# Autodesk Inventor assembly: WCP-0897
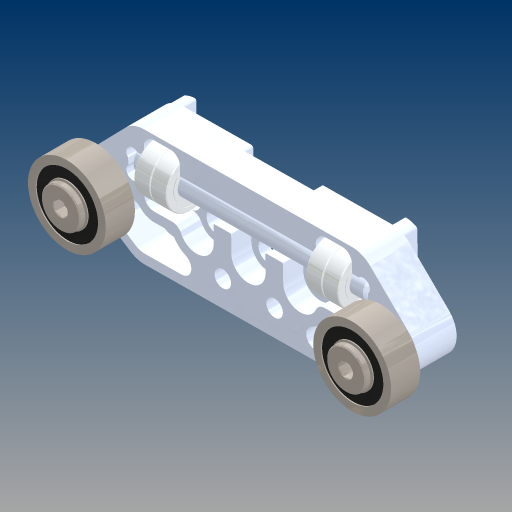
[picture p0: Inventor's stored thumbnail of the model, 512x512]
Saved by Autodesk Inventor 2024.3 (Build 283343000, 343)
## iProperties
Created: 2023-01-17
Part Number: WCP-0897
Description: STEP AP214
Document SubType Name: Assembly
Designer: Kenji
Title: WCP-0897.step
Revision Number: ANY
Sending System: SolidWorks 2020
Preprocessor: SwSTEP 2.0
## Documents named in this file (6)
- C:\Users\Kenji\Documents\GitHub\1622-2024-Casino-Clash-CAD-A-Thon\COTS Library\Motion\BearingBlocks\ElevatorBlocks\WCP-0897_InlineBearingBlock.iam
- C:\Users\Kenji\Downloads\WCP-0897 (1)\WCP-0897 (1)\WCP-0897-001 Rev1.ipt
- C:\Users\Kenji\Downloads\WCP-0897 (1)\WCP-0897 (1)\WCP-0897-002 Rev1.ipt
- C:\Users\Kenji\Downloads\WCP-0897 (1)\WCP-0897 (1)\WCP-0498 Rev1.ipt
- C:\Users\Kenji\Downloads\WCP-0897 (1)\WCP-0897 (1)\WCP-0473 Rev1.ipt
- C:\Users\Kenji\Downloads\WCP-0897 (1)\WCP-0897 (1)\WCP-0212_0_250_radial_bearing.ipt
## Components (10 placed, 10 different names)
1. WCP-0897-001 Rev1_1 — Mate:9, Mate:10, Mate:13, Mate:14, Tangent:1, Tangent:2, Mate:15, Mate:16, Mate:17
2. WCP-0897-002 Rev1_2 — Mate:1, Mate:2, Mate:4, Mate:5, Tangent:1, Tangent:2, Mate:17
3. WCP-0498 Rev1_3 — Mate:5, Mate:6, Mate:16
4. WCP-0498 Rev1_4 — Mate:4, Mate:6
5. WCP-0498 Rev1_5 — Mate:2, Mate:3, Mate:15
6. WCP-0498 Rev1_6 — Mate:1, Mate:3
7. WCP-0473 Rev1_7 — Mate:11, Mate:12, Mate:14
8. WCP-0473 Rev1_8 — Mate:7, Mate:8, Mate:10
9. WCP-0212_0_250_radial_bearing_9 — Mate:11, Mate:12, Mate:13
10. WCP-0212_0_250_radial_bearing_10 — Mate:7, Mate:8, Mate:9
## Relationships (19: Mate 17, Tangent 2)
- Mate:1: WCP-0897-002 Rev1_2 ↔ WCP-0498 Rev1_6
- Mate:2: WCP-0897-002 Rev1_2 ↔ WCP-0498 Rev1_5
- Mate:3: WCP-0498 Rev1_5 ↔ WCP-0498 Rev1_6
- Mate:4: WCP-0897-002 Rev1_2 ↔ WCP-0498 Rev1_4
- Mate:5: WCP-0897-002 Rev1_2 ↔ WCP-0498 Rev1_3
- Mate:6: WCP-0498 Rev1_3 ↔ WCP-0498 Rev1_4
- Mate:7: WCP-0473 Rev1_8 ↔ WCP-0212_0_250_radial_bearing_10
- Mate:8: WCP-0473 Rev1_8 ↔ WCP-0212_0_250_radial_bearing_10
- Mate:9: WCP-0897-001 Rev1_1 ↔ WCP-0212_0_250_radial_bearing_10
- Mate:10: WCP-0897-001 Rev1_1 ↔ WCP-0473 Rev1_8
- Mate:11: WCP-0473 Rev1_7 ↔ WCP-0212_0_250_radial_bearing_9
- Mate:12: WCP-0473 Rev1_7 ↔ WCP-0212_0_250_radial_bearing_9
- Mate:13: WCP-0897-001 Rev1_1 ↔ WCP-0212_0_250_radial_bearing_9
- Mate:14: WCP-0897-001 Rev1_1 ↔ WCP-0473 Rev1_7
- Tangent:1: WCP-0897-001 Rev1_1 ↔ WCP-0897-002 Rev1_2
- Tangent:2: WCP-0897-001 Rev1_1 ↔ WCP-0897-002 Rev1_2
- Mate:15 (0.4191 mm): WCP-0897-001 Rev1_1 ↔ WCP-0498 Rev1_5
- Mate:16 (0.4191 mm): WCP-0897-001 Rev1_1 ↔ WCP-0498 Rev1_3
- Mate:17 (0.8001 mm): WCP-0897-001 Rev1_1 ↔ WCP-0897-002 Rev1_2
